# Autodesk Inventor assembly: bepf_platforma
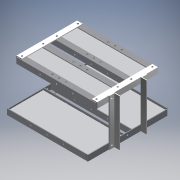
[picture p0: Inventor's stored thumbnail of the model, 180x180]
Saved by Autodesk Inventor 2017 (Build 210142000, 142)
## iProperties
Part Number: bepf_platforma
Material: Ogólny
Document SubType Name: Assembly
Designer: gagato
Author: gagato
## Documents named in this file (4)
- C:\Users\gagato\Documents\bepf\bepf_platforma.iam
- C:\Users\gagato\Documents\bepf\bepf_platforma_polka_dolna.iam
- C:\Users\gagato\Documents\bepf\bepf_platforma_rama_lacznik_pionowy.ipt
- C:\Users\gagato\Documents\bepf\bepf_platforma_polka_gorna.iam
## Components (4 placed, 3 different names)
1. bepf_platforma_polka_dolna:1 [sub-assembly] — Zestawiający:1, Zestawiający:2, Zestawiający:3, Zestawiający:4, Równoległy:1, Równoległy:2, Zestawiający:8
2. bepf_platforma_rama_lacznik_pionowy:1 — Zestawiający:1, Zestawiający:2, Równoległy:1, Zestawiający:7
3. bepf_platforma_rama_lacznik_pionowy:2 — Zestawiający:3, Zestawiający:4, Równoległy:2, Zestawiający:5, Zestawiający:6
4. bepf_platforma_polka_gorna:1 [sub-assembly] — Zestawiający:5, Zestawiający:6, Zestawiający:7
## Relationships (10: Mate 8, Flush 2)
- Zestawiający:1 [Mate]: bepf_platforma_polka_dolna:1 ↔ bepf_platforma_rama_lacznik_pionowy:1
- Zestawiający:2 [Mate]: bepf_platforma_polka_dolna:1 ↔ bepf_platforma_rama_lacznik_pionowy:1
- Zestawiający:3 [Mate]: bepf_platforma_polka_dolna:1 ↔ bepf_platforma_rama_lacznik_pionowy:2
- Zestawiający:4 [Mate]: bepf_platforma_polka_dolna:1 ↔ bepf_platforma_rama_lacznik_pionowy:2
- Równoległy:1 [Flush]: bepf_platforma_polka_dolna:1 ↔ bepf_platforma_rama_lacznik_pionowy:1
- Równoległy:2 [Flush]: bepf_platforma_polka_dolna:1 ↔ bepf_platforma_rama_lacznik_pionowy:2
- Zestawiający:5 [Mate]: bepf_platforma_rama_lacznik_pionowy:2 ↔ bepf_platforma_polka_gorna:1
- Zestawiający:6 [Mate]: bepf_platforma_rama_lacznik_pionowy:2 ↔ bepf_platforma_polka_gorna:1
- Zestawiający:7 [Mate]: bepf_platforma_rama_lacznik_pionowy:1 ↔ bepf_platforma_polka_gorna:1
- Zestawiający:8 [Mate]: bepf_platforma_polka_dolna:1
